# Autodesk Inventor assembly: WheelNGear
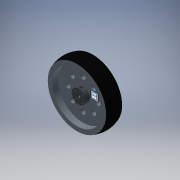
[picture p0: Inventor's stored thumbnail of the model, 180x180]
Saved by Autodesk Inventor 2016 (Build 200138000, 138)
## iProperties
Created: 2015-08-30
Part Number: WheelNGear
Document SubType Name: Assembly
Designer: Tim
Author: Tim
## Documents named in this file (5)
- C:\Users\Tim\Documents\GitHub\phi_robotics\3d-models\FTC_Tetrix_KOP_Block_Party\WheelNGear.iam
- C:\Users\Tim\Documents\GitHub\phi_robotics\3d-models\FTC_Tetrix_KOP_Block_Party\Tetrix_Kit_FTC\Autodesk Inventor Files\tetrix_wheel.ipt
- C:\Users\Tim\Documents\GitHub\phi_robotics\3d-models\FTC_Tetrix_KOP_Block_Party\Tetrix_Kit_FTC\Autodesk Inventor Files\tetrix_gear-med.ipt
- C:\Users\Tim\Documents\GitHub\phi_robotics\3d-models\FTC_Tetrix_KOP_Block_Party\Tetrix_Kit_FTC\Autodesk Inventor Files\tetrix_axle_lock.iam
- C:\Users\Tim\Documents\GitHub\phi_robotics\3d-models\FTC_Tetrix_KOP_Block_Party\Tetrix_Kit_FTC\Autodesk Inventor Files\tetrix_axle_spacer_mount.ipt
## Components (5 placed, 4 different names)
1. tetrix_wheel:1 — Rigid:1, Rigid:4
2. tetrix_gear-med:1 — Rigid:2, Rigid:3
3. tetrix_axle_lock:1 [sub-assembly] — Rigid:4
4. tetrix_axle_lock:2 [sub-assembly] — Rigid:3
5. tetrix_axle_spacer_mount:1 — Rigid:1, Rigid:2
## Relationships (4: WeldJoint 4)
- Rigid:1 [WeldJoint]: tetrix_wheel:1 ↔ tetrix_axle_spacer_mount:1
- Rigid:2 [WeldJoint]: tetrix_gear-med:1 ↔ tetrix_axle_spacer_mount:1
- Rigid:3 [WeldJoint]: tetrix_gear-med:1 ↔ tetrix_axle_lock:2
- Rigid:4 [WeldJoint]: tetrix_wheel:1 ↔ tetrix_axle_lock:1
